# Autodesk Inventor assembly: Arm Assembly
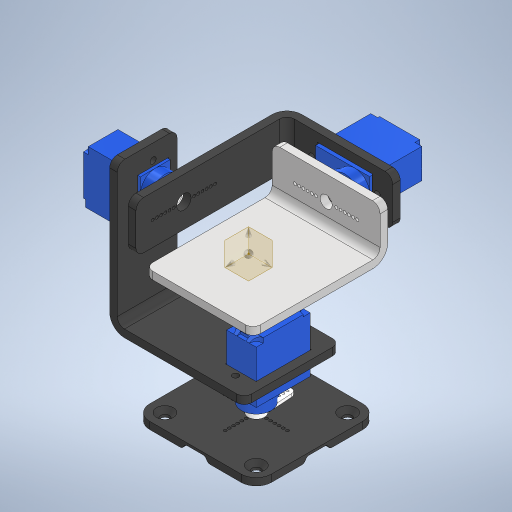
[picture p0: Inventor's stored thumbnail of the model, 512x512]
Saved by Autodesk Inventor 2023.4 (Build 274418000, 418)
## iProperties
Created: 2024-05-24
Part Number: Arm Assembly
Document SubType Name: Assembly
Designer: Nathan Cai
Author: Nathan Cai
## Documents named in this file (7)
- E:\Documents\Inventor\Arduino - Gimble\Arm Assembly.iam
- E:\Documents\Inventor\Arduino - Gimble\Base.ipt
- E:\Documents\Inventor\Arduino - Gimble\Servohorn\Servohorn.ipt
- E:\Documents\Inventor\Arduino - Gimble\Servo SG90\Servo SG90.ipt
- E:\Documents\Inventor\Arduino - Gimble\Midplate.ipt
- E:\Documents\Inventor\Arduino - Gimble\Topplate.ipt
- E:\Documents\Inventor\Arduino - Gimble\Platform.ipt
## Components (10 placed, 6 different names)
1. Base:1 — Mate:1, Mate:2, Mate:3
2. Servohorn:1 — Mate:1, Mate:2, Mate:3, Mate:4, Mate:5
3. Servo SG90:1 — Mate:4, Mate:5, Mate:6, Mate:7, Mate:8
4. Midplate:1 — Mate:6, Mate:7, Mate:8, Mate:9, Mate:10, Mate:11
5. Servo SG90:2 — Mate:9, Mate:10, Mate:11, Mate:12, Mate:13
6. Servohorn:2 — Mate:12, Mate:13, Mate:14, Mate:15, Mate:16
7. Topplate:1 — Mate:14, Mate:15, Mate:16, Mate:17, Mate:18, Mate:19
8. Servo SG90:3 — Mate:17, Mate:18, Mate:19, Mate:20, Mate:21
9. Servohorn:3 — Mate:20, Mate:21, Mate:22, Mate:23, Mate:24
10. Platform:1 — Mate:22, Mate:23, Mate:24
## Relationships (24: Mate 24)
- Mate:1: Base:1 ↔ Servohorn:1
- Mate:2: Base:1 ↔ Servohorn:1
- Mate:3: Base:1 ↔ Servohorn:1
- Mate:4: Servohorn:1 ↔ Servo SG90:1
- Mate:5: Servohorn:1 ↔ Servo SG90:1
- Mate:6: Servo SG90:1 ↔ Midplate:1
- Mate:7: Servo SG90:1 ↔ Midplate:1
- Mate:8: Servo SG90:1 ↔ Midplate:1
- Mate:9: Midplate:1 ↔ Servo SG90:2
- Mate:10: Midplate:1 ↔ Servo SG90:2
- Mate:11: Midplate:1 ↔ Servo SG90:2
- Mate:12: Servo SG90:2 ↔ Servohorn:2
- Mate:13: Servo SG90:2 ↔ Servohorn:2
- Mate:14: Servohorn:2 ↔ Topplate:1
- Mate:15: Servohorn:2 ↔ Topplate:1
- Mate:16: Servohorn:2 ↔ Topplate:1
- Mate:17: Topplate:1 ↔ Servo SG90:3
- Mate:18: Topplate:1 ↔ Servo SG90:3
- Mate:19: Topplate:1 ↔ Servo SG90:3
- Mate:20: Servo SG90:3 ↔ Servohorn:3
- Mate:21: Servo SG90:3 ↔ Servohorn:3
- Mate:22: Servohorn:3 ↔ Platform:1
- Mate:23: Servohorn:3 ↔ Platform:1
- Mate:24: Servohorn:3 ↔ Platform:1
